# Autodesk Inventor assembly: sensor_box
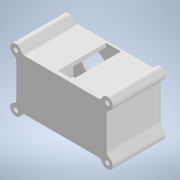
[picture p0: Inventor's stored thumbnail of the model, 180x180]
Saved by Autodesk Inventor 2020 (Build 240168000, 168)
## iProperties
Created: 2020-03-10
Part Number: sensor_box
Document SubType Name: Assembly
Designer: Richard
Author: Richard
## Documents named in this file (3)
- F:\Richard\Documents\psu\OpenZ\3d_STLs\SENSOR\sensor_box.iam
- F:\Richard\Documents\psu\OpenZ\3d_STLs\SENSOR\sensor_housing.ipt
- F:\Richard\Documents\psu\OpenZ\3d_STLs\SENSOR\sensor_lid.ipt
## Components (2 placed, 2 different names)
1. sensor_housing:1 — Mate:1, Insert:1, Insert:2
2. sensor_lid:1 — Mate:1, Insert:1, Insert:2
## Relationships (3: Insert 2, Mate 1)
- Mate:1: sensor_housing:1 ↔ sensor_lid:1
- Insert:1: sensor_housing:1 ↔ sensor_lid:1
- Insert:2: sensor_housing:1 ↔ sensor_lid:1
